# Autodesk Inventor assembly: Assembly
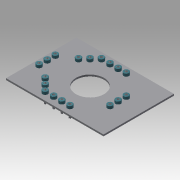
[picture p0: Inventor's stored thumbnail of the model, 180x180]
Saved by Autodesk Inventor 2019.3 (Build 233278000, 278)
## iProperties
Created: 2019-03-22
Part Number: Assembly
Document SubType Name: Assembly
Designer: Dave
Author: Dave
## Documents named in this file (3)
- C:\Users\Dave\Dropbox\ProjectODMeter\HousingCAD\Assembly.iam
- C:\Users\Dave\Dropbox\ProjectODMeter\HousingCAD\banana_plug_recepticle.ipt
- C:\Users\Dave\Dropbox\ProjectODMeter\HousingCAD\top_plate.ipt
## Components (19 placed, 2 different names)
1. banana_plug_recepticle:1 — Mate:3, Mate:19
2. top_plate:1 — Mate:1, Mate:2, Mate:3, Mate:4, Mate:5, Mate:6, Mate:7, Mate:8, Mate:9, Mate:10, Mate:11, Mate:12, Mate:13, Mate:14, Mate:15, Mate:16, Mate:17, Mate:18, Mate:19, Mate:20, Mate:21, Mate:22, Mate:23, Mate:24, Mate:25, Mate:26, Mate:27, Mate:28, Mate:29, Mate:30, Mate:31, Mate:32, Mate:33, Mate:34, Mate:35, Mate:36
3. banana_plug_recepticle:2 — Mate:1, Mate:21
4. banana_plug_recepticle:3 — Mate:2, Mate:20
5. banana_plug_recepticle:4 — Mate:4, Mate:36
6. banana_plug_recepticle:5 — Mate:5, Mate:35
7. banana_plug_recepticle:6 — Mate:8, Mate:32
8. banana_plug_recepticle:7 — Mate:6, Mate:34
9. banana_plug_recepticle:8 — Mate:7, Mate:33
10. banana_plug_recepticle:9 — Mate:14, Mate:26
11. banana_plug_recepticle:10 — Mate:12, Mate:28
12. banana_plug_recepticle:11 — Mate:13, Mate:27
13. banana_plug_recepticle:12 — Mate:15, Mate:25
14. banana_plug_recepticle:13 — Mate:11, Mate:29
15. banana_plug_recepticle:14 — Mate:10, Mate:30
16. banana_plug_recepticle:15 — Mate:9, Mate:31
17. banana_plug_recepticle:16 — Mate:16, Mate:24
18. banana_plug_recepticle:17 — Mate:17, Mate:23
19. banana_plug_recepticle:18 — Mate:18, Mate:22
## Relationships (36: Mate 36)
- Mate:1: top_plate:1 ↔ banana_plug_recepticle:2
- Mate:2: top_plate:1 ↔ banana_plug_recepticle:3
- Mate:3: banana_plug_recepticle:1 ↔ top_plate:1
- Mate:4: top_plate:1 ↔ banana_plug_recepticle:4
- Mate:5: top_plate:1 ↔ banana_plug_recepticle:5
- Mate:6: top_plate:1 ↔ banana_plug_recepticle:7
- Mate:7: top_plate:1 ↔ banana_plug_recepticle:8
- Mate:8: top_plate:1 ↔ banana_plug_recepticle:6
- Mate:9: top_plate:1 ↔ banana_plug_recepticle:15
- Mate:10: top_plate:1 ↔ banana_plug_recepticle:14
- Mate:11: top_plate:1 ↔ banana_plug_recepticle:13
- Mate:12: top_plate:1 ↔ banana_plug_recepticle:10
- Mate:13: top_plate:1 ↔ banana_plug_recepticle:11
- Mate:14: top_plate:1 ↔ banana_plug_recepticle:9
- Mate:15: top_plate:1 ↔ banana_plug_recepticle:12
- Mate:16: top_plate:1 ↔ banana_plug_recepticle:16
- Mate:17: top_plate:1 ↔ banana_plug_recepticle:17
- Mate:18: top_plate:1 ↔ banana_plug_recepticle:18
- Mate:19: banana_plug_recepticle:1 ↔ top_plate:1
- Mate:20: top_plate:1 ↔ banana_plug_recepticle:3
- Mate:21: top_plate:1 ↔ banana_plug_recepticle:2
- Mate:22: top_plate:1 ↔ banana_plug_recepticle:18
- Mate:23: top_plate:1 ↔ banana_plug_recepticle:17
- Mate:24: top_plate:1 ↔ banana_plug_recepticle:16
- Mate:25: top_plate:1 ↔ banana_plug_recepticle:12
- Mate:26: top_plate:1 ↔ banana_plug_recepticle:9
- Mate:27: top_plate:1 ↔ banana_plug_recepticle:11
- Mate:28: top_plate:1 ↔ banana_plug_recepticle:10
- Mate:29: top_plate:1 ↔ banana_plug_recepticle:13
- Mate:30: top_plate:1 ↔ banana_plug_recepticle:14
- Mate:31: top_plate:1 ↔ banana_plug_recepticle:15
- Mate:32: top_plate:1 ↔ banana_plug_recepticle:6
- Mate:33: top_plate:1 ↔ banana_plug_recepticle:8
- Mate:34: top_plate:1 ↔ banana_plug_recepticle:7
- Mate:35: top_plate:1 ↔ banana_plug_recepticle:5
- Mate:36: top_plate:1 ↔ banana_plug_recepticle:4
